# Autodesk Inventor assembly: !Arm
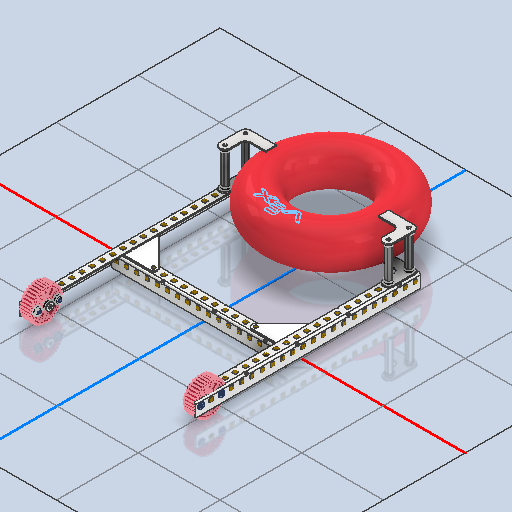
[picture p0: Inventor's stored thumbnail of the model, 512x512]
Saved by Autodesk Inventor 2026 (Build 300175000, 175)
## iProperties
Created: 2025-04-06
Part Number: !Arm
Document SubType Name: Assembly
Designer: avere
Author: avere
## Documents named in this file (24)
- C:\Users\avere\OneDrive\Documents\VEX-CAD\V5-CAD\Lady Brown\Arm\!Arm.iam
- C:\Users\avere\OneDrive\Documents\VEX-CAD\VEX-CAD-Inventor\Structure\C Channel\Aluminum 1x3x1 Half Thick Cut\Alu C Half Thick 1x3x1x22.ipt
- C:\Users\avere\OneDrive\Documents\VEX-CAD\VEX-CAD-Inventor\Motion\Gears\HS Gear\HS 36T Gear, No Insert.iam
- C:\Users\avere\OneDrive\Documents\VEX-CAD\VEX-CAD-Inventor\Motion\Gears\HS Gear.iam
- C:\Users\avere\OneDrive\Documents\VEX-CAD\VEX-CAD-Inventor\Structure\Hardware\Screw Steel - Star\SScrew Star Smooth .750.ipt
- C:\Users\avere\OneDrive\Documents\VEX-CAD\VEX-CAD-Inventor\Structure\Hardware\Screw Steel - Star.ipt
- C:\Users\avere\OneDrive\Documents\VEX-CAD\VEX-CAD-Inventor\Structure\Hardware\Nut Nylon\Nut Nylon - Black.ipt
- C:\Users\avere\OneDrive\Documents\VEX-CAD\VEX-CAD-Inventor\Structure\Hardware\Nut Nylon.ipt
- C:\Users\avere\OneDrive\Documents\VEX-CAD\V5-CAD\Lady Brown\Arm\Alu C Half Thick 1x3x1x22 Mirrored.ipt
- C:\Users\avere\OneDrive\Documents\VEX-CAD\VEX-CAD-Inventor\Structure\C Channel\Aluminum 1x3x1 Half Thick Cut\Alu C Half Thick 1x3x1x17.ipt
- C:\Users\avere\OneDrive\Documents\VEX-CAD\V5-CAD\Lady Brown\Arm\Custom Parts\Triangle Gusset.ipt
- C:\Users\avere\OneDrive\Documents\VEX-CAD\V5-CAD\Lady Brown\Arm\Custom Parts\Magazine Gusset.ipt
- C:\Users\avere\OneDrive\Documents\VEX-CAD\VEX-CAD-Inventor\Structure\Standoff.ipt
- C:\Users\avere\OneDrive\Documents\VEX-CAD\V5-CAD\Lady Brown\Arm\Custom Parts\Magazine Gusset mirrored.ipt
- C:\Users\avere\OneDrive\Documents\VEX-CAD\VEX-CAD-Inventor\Motion\Spacers\Washer Teflon\TWasher .375 OD x .03125.ipt
- C:\Users\avere\OneDrive\Documents\VEX-CAD\VEX-CAD-Inventor\Motion\Spacers\Washer Teflon.ipt
- C:\Users\avere\OneDrive\Documents\VEX-CAD\VEX-CAD-Inventor\Motion\Spacers\Washer Steel\SWasher .375 OD x .015625.ipt
- C:\Users\avere\OneDrive\Documents\VEX-CAD\VEX-CAD-Inventor\Motion\Spacers\Washer Steel.ipt
- C:\Users\avere\OneDrive\Documents\VEX-CAD\VEX-CAD-Inventor\Motion\Spacers\Spacer Nylon .375 OD\NSpacer .375 OD x .375.ipt
- C:\Users\avere\OneDrive\Documents\VEX-CAD\VEX-CAD-Inventor\Motion\Spacers\Spacer Nylon .375 OD.ipt
- C:\Users\avere\OneDrive\Documents\VEX-CAD\VEX-CAD-Inventor\Motion\Spacers\Spacer Nylon .375 OD\NSpacer .375 OD x .125.ipt
- C:\Users\avere\OneDrive\Documents\VEX-CAD\VEX-CAD-Inventor\Motion\Spacers\Washer Teflon\TWasher .375 OD x .04000.ipt
- C:\Users\avere\OneDrive\Documents\VEX-CAD\VEX-CAD-Inventor\Game Objects\High Stakes\Rings\Red Ring.ipt
- C:\Users\avere\OneDrive\Documents\VEX-CAD\VEX-CAD-Inventor\Structure\Standoff\Standoff 1.50.ipt
## Components (38 placed, 16 different names)
1. Alu C Half Thick 1x3x1x22:1 — Mate:1, Mate:2, Flush:1, Insert:1, Mate:3, Angle:1, Insert:2, Mate:7, Insert:25, Mate:12
2. HS 36T Gear, No Insert:1 [sub-assembly] — Insert:1, Mate:3, Insert:3, Insert:21
3. Alu C Half Thick 1x3x1x22 Mirrored:1 — Angle:2, Flush:2, Mate:4, Mate:5, Mate:6, Insert:4, Insert:5, Insert:7, Insert:8, Insert:40, Mate:14
4. HS 36T Gear, No Insert:2 [sub-assembly] — Mate:6, Insert:4, Insert:6, Insert:24
5. Alu C Half Thick 1x3x1x17:1 — Insert:7, Mate:7, Mate:8
6. Triangle Gusset:1 — Insert:8, Mate:8
7. Triangle Gusset:2
8. Magazine Gusset:1 — Mate:11, Insert:26
9. Magazine Gusset:2 — Insert:25, Mate:12, Insert:26, Insert:31, Insert:32
10. Magazine Gusset mirrored:1 — Insert:39, Mate:13
11. Magazine Gusset mirrored:2 — Insert:35, Insert:38, Insert:40, Mate:14
12. TWasher .375 OD x .03125:1 — Insert:19, Insert:20
13. SWasher .375 OD x .015625:1 — Insert:19
14. NSpacer .375 OD x .375:1 — Insert:20, Insert:21
15. TWasher .375 OD x .03125:2 — Insert:22
16. NSpacer .375 OD x .125:2 — Insert:23, Insert:24
17. TWasher .375 OD x .04000:3 — Insert:22, Insert:23
18. Red Ring:1 — Mate:9, Mate:10, Mate:11
19. Standoff 1.50:9 — Insert:27, Insert:28
20. NSpacer .375 OD x .125:3 — Insert:27
21. NSpacer .375 OD x .125:4 — Insert:28, Insert:31
22. Standoff 1.50:10
23. NSpacer .375 OD x .125:5
24. NSpacer .375 OD x .125:6 — Insert:32
25. Standoff 1.50:11
26. NSpacer .375 OD x .125:7 — Insert:35
27. NSpacer .375 OD x .125:8 — Mate:13
28. Standoff 1.50:12
29. NSpacer .375 OD x .125:9 — Insert:38
30. NSpacer .375 OD x .125:10 — Insert:39
31. SScrew Star Smooth .750:1 — Insert:2
32. Nut Nylon - Black:1 — Insert:3
33. SScrew Star Smooth .750:2
34. Nut Nylon - Black:2
35. SScrew Star Smooth .750:3 — Insert:5
36. Nut Nylon - Black:3 — Insert:6
37. SScrew Star Smooth .750:4
38. Nut Nylon - Black:4
## Component patterns: (2 elements, first: SScrew Star Smooth .750:1 + Nut Nylon - Black:1), (2 elements, first: SScrew Star Smooth .750:3 + Nut Nylon - Black:3)
## Relationships (48: Insert 30, Mate 14, Flush 2, Angle 2)
- Mate:1 (101.6 mm): Alu C Half Thick 1x3x1x22:1
- Mate:2: Alu C Half Thick 1x3x1x22:1
- Flush:1 (-139.7 mm): Alu C Half Thick 1x3x1x22:1
- Insert:1: Alu C Half Thick 1x3x1x22:1 ↔ HS 36T Gear, No Insert:1
- Mate:3: Alu C Half Thick 1x3x1x22:1 ↔ HS 36T Gear, No Insert:1
- Angle:1 (0 deg): Alu C Half Thick 1x3x1x22:1
- Insert:2: Alu C Half Thick 1x3x1x22:1 ↔ SScrew Star Smooth .750:1
- Insert:3: HS 36T Gear, No Insert:1 ↔ Nut Nylon - Black:1
- Angle:2 (0 deg): Alu C Half Thick 1x3x1x22 Mirrored:1
- Flush:2 (-139.7 mm): Alu C Half Thick 1x3x1x22 Mirrored:1
- Mate:4: Alu C Half Thick 1x3x1x22 Mirrored:1
- Mate:5 (-101.6 mm): Alu C Half Thick 1x3x1x22 Mirrored:1
- Mate:6: Alu C Half Thick 1x3x1x22 Mirrored:1 ↔ HS 36T Gear, No Insert:2
- Insert:4: Alu C Half Thick 1x3x1x22 Mirrored:1 ↔ HS 36T Gear, No Insert:2
- Insert:5: Alu C Half Thick 1x3x1x22 Mirrored:1 ↔ SScrew Star Smooth .750:3
- Insert:6: HS 36T Gear, No Insert:2 ↔ Nut Nylon - Black:3
- Insert:7 (1.5875 mm): Alu C Half Thick 1x3x1x22 Mirrored:1 ↔ Alu C Half Thick 1x3x1x17:1
- Mate:7: Alu C Half Thick 1x3x1x22:1 ↔ Alu C Half Thick 1x3x1x17:1
- Insert:8: Alu C Half Thick 1x3x1x22 Mirrored:1 ↔ Triangle Gusset:1
- Mate:8: Alu C Half Thick 1x3x1x17:1 ↔ Triangle Gusset:1
- Insert:19: TWasher .375 OD x .03125:1 ↔ SWasher .375 OD x .015625:1
- Insert:20: TWasher .375 OD x .03125:1 ↔ NSpacer .375 OD x .375:1
- Insert:21: HS 36T Gear, No Insert:1 ↔ NSpacer .375 OD x .375:1
- Insert:22: TWasher .375 OD x .03125:2 ↔ TWasher .375 OD x .04000:3
- Insert:23: NSpacer .375 OD x .125:2 ↔ TWasher .375 OD x .04000:3
- Insert:24: HS 36T Gear, No Insert:2 ↔ NSpacer .375 OD x .125:2
- Mate:9: Red Ring:1
- Mate:10 (28.575 mm): Red Ring:1
- Mate:11: Magazine Gusset:1 ↔ Red Ring:1
- Insert:25: Alu C Half Thick 1x3x1x22:1 ↔ Magazine Gusset:2
- Mate:12: Alu C Half Thick 1x3x1x22:1 ↔ Magazine Gusset:2
- Insert:26 (44.45 mm): Magazine Gusset:1 ↔ Magazine Gusset:2
- Insert:27: Standoff 1.50:9 ↔ NSpacer .375 OD x .125:3
- Insert:28: Standoff 1.50:9 ↔ NSpacer .375 OD x .125:4
- [Insert]: Standoff 1.50:10 ↔ NSpacer .375 OD x .125:5
- [Insert]: Standoff 1.50:10 ↔ NSpacer .375 OD x .125:6
- Insert:31: Magazine Gusset:2 ↔ NSpacer .375 OD x .125:4
- Insert:32: Magazine Gusset:2 ↔ NSpacer .375 OD x .125:6
- [Insert]: Standoff 1.50:11 ↔ NSpacer .375 OD x .125:7
- [Insert]: Standoff 1.50:11 ↔ NSpacer .375 OD x .125:8
- Insert:35: Magazine Gusset mirrored:2 ↔ NSpacer .375 OD x .125:7
- [Insert]: Standoff 1.50:12 ↔ NSpacer .375 OD x .125:9
- [Insert]: Standoff 1.50:12 ↔ NSpacer .375 OD x .125:10
- Insert:38: Magazine Gusset mirrored:2 ↔ NSpacer .375 OD x .125:9
- Insert:39: Magazine Gusset mirrored:1 ↔ NSpacer .375 OD x .125:10
- Mate:13: Magazine Gusset mirrored:1 ↔ NSpacer .375 OD x .125:8
- Insert:40: Alu C Half Thick 1x3x1x22 Mirrored:1 ↔ Magazine Gusset mirrored:2
- Mate:14: Alu C Half Thick 1x3x1x22 Mirrored:1 ↔ Magazine Gusset mirrored:2
## Named parameters: d66_d64 = 0 mm, d67_d65 = 0 mm, d70_d64 = 0 mm, d71_d65 = 0 mm, d73_d64 = 0 mm, d74_d65 = 0 mm
